# Autodesk Inventor assembly: Assembly - FixedV2
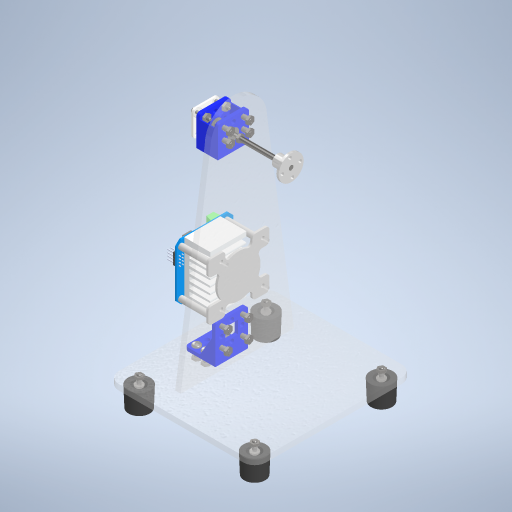
[picture p0: Inventor's stored thumbnail of the model, 512x512]
Saved by Autodesk Inventor 2023.1 (Build 271208000, 208)
## iProperties
Created: 2023-05-11
Part Number: Assembly - FixedV2
Document SubType Name: Assembly
Designer: felip
Author: felip
## Documents named in this file (4)
- C:\Users\felip\OneDrive\UNAL FORE\SEMESTRE 9\TECNICAS DE CONTROL\PROYECTO\PROYECTO-TDC-INVENTOR\Assembly - FixedV2.iam
- C:\Users\felip\OneDrive\UNAL FORE\SEMESTRE 9\TECNICAS DE CONTROL\PROYECTO\PROYECTO-TDC-INVENTOR\BTS7960 43A HIGH POWER H BRIDGE MODULE.iam
- C:\Users\felip\OneDrive\UNAL FORE\SEMESTRE 9\TECNICAS DE CONTROL\PROYECTO\PROYECTO-TDC-INVENTOR\Assembly - Fixed.iam
- C:\Users\felip\OneDrive\UNAL FORE\SEMESTRE 9\TECNICAS DE CONTROL\PROYECTO\PROYECTO-TDC-INVENTOR\soporteHBridge.ipt
## Components (3 placed, 3 different names)
1. Assembly - Fixed:1 [sub-assembly] — Mate:2, Flush:1, Flush:2, Flush:3
2. BTS7960 43A HIGH POWER H BRIDGE MODULE:1 [sub-assembly] — Mate:2, Flush:1, Mate:3
3. soporteHBridge:1 — Flush:2, Flush:3, Mate:3
## Relationships (5: Flush 3, Mate 2)
- Mate:2 (35 mm): Assembly - Fixed:1 ↔ BTS7960 43A HIGH POWER H BRIDGE MODULE:1
- Flush:1 (-6 mm): Assembly - Fixed:1 ↔ BTS7960 43A HIGH POWER H BRIDGE MODULE:1
- Flush:2: Assembly - Fixed:1 ↔ soporteHBridge:1
- Flush:3: Assembly - Fixed:1 ↔ soporteHBridge:1
- Mate:3: BTS7960 43A HIGH POWER H BRIDGE MODULE:1 ↔ soporteHBridge:1
